# Autodesk Inventor assembly: TabletMountAssembly
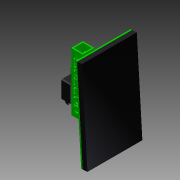
[picture p0: Inventor's stored thumbnail of the model, 180x180]
Saved by Autodesk Inventor 2012 (Build 160160000, 160)
## iProperties
Created: 2013-10-06
Part Number: TabletMountAssembly
Document SubType Name: Assembly
Designer: joe_000
Author: joe_000
## Documents named in this file (8)
- C:\dev\telepresenceRobot\mechanical\TabletMountAssembly.iam
- C:\dev\telepresenceRobot\mechanical\Nexus7.ipt
- C:\dev\telepresenceRobot\mechanical\TableMount-Holder.ipt
- C:\dev\telepresenceRobot\mechanical\Servo.ipt
- C:\dev\telepresenceRobot\mechanical\Servo-Horn.ipt
- C:\dev\telepresenceRobot\mechanical\TabletMount-ServoWire.ipt
- C:\dev\telepresenceRobot\mechanical\TabletMount-Mast-Right.ipt
- C:\dev\telepresenceRobot\mechanical\TabletMount-Mast-Left.ipt
## Components (7 placed, 7 different names)
1. TabletMount-Mast-Right:1 — Mate:6, Insert:5, Insert:6, Flush:11, Mate:7, Flush:12, Mate:8, Insert:7
2. Nexus7:1 — Mate:5, Flush:9, Flush:10
3. TableMount-Holder:1 — Mate:5, Flush:9, Flush:10, Mate:8, Insert:7, Tangent:1
4. Servo:1 — Insert:3, Mate:6, Insert:5, Insert:6
5. Servo-Horn:1 — Insert:3, Insert:4
6. TabletMount-ServoWire:1 — Insert:4, Tangent:1
7. TabletMount-Mast-Left:1 — Flush:11, Mate:7, Flush:12
## Relationships (14: Insert 5, Mate 4, Flush 4, Tangent 1)
- Mate:5: Nexus7:1 ↔ TableMount-Holder:1
- Flush:9: Nexus7:1 ↔ TableMount-Holder:1
- Flush:10: Nexus7:1 ↔ TableMount-Holder:1
- Insert:3: Servo:1 ↔ Servo-Horn:1
- Insert:4: Servo-Horn:1 ↔ TabletMount-ServoWire:1
- Mate:6: TabletMount-Mast-Right:1 ↔ Servo:1
- Insert:5: TabletMount-Mast-Right:1 ↔ Servo:1
- Insert:6: TabletMount-Mast-Right:1 ↔ Servo:1
- Flush:11: TabletMount-Mast-Right:1 ↔ TabletMount-Mast-Left:1
- Mate:7: TabletMount-Mast-Right:1 ↔ TabletMount-Mast-Left:1
- Flush:12: TabletMount-Mast-Right:1 ↔ TabletMount-Mast-Left:1
- Mate:8: TabletMount-Mast-Right:1 ↔ TableMount-Holder:1
- Insert:7: TabletMount-Mast-Right:1 ↔ TableMount-Holder:1
- Tangent:1: TableMount-Holder:1 ↔ TabletMount-ServoWire:1
